# Autodesk Inventor assembly: Swerve-Drivetrain-2
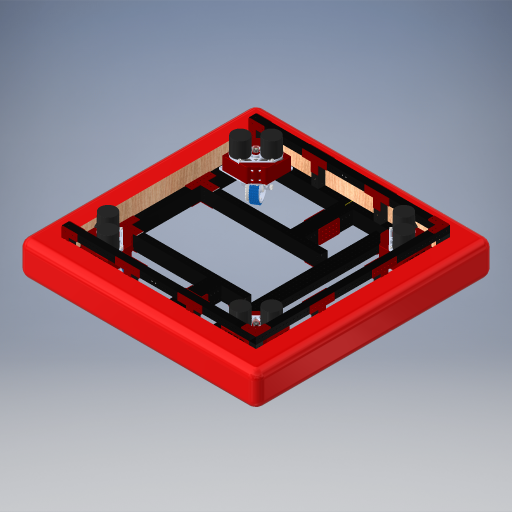
[picture p0: Inventor's stored thumbnail of the model, 512x512]
Saved by Autodesk Inventor 2024.2 (Build 282272000, 272)
## iProperties
Created: 2024-01-06
Part Number: Swerve-Drivetrain-2
Document SubType Name: Assembly
Designer: rohan
Author: rohan
## Documents named in this file (15)
- C:\Users\rohan\OneDrive - Hillsborough County Public Schools\Robotics\FIRST-Robotics-Competition\Crescendo\Minotaur-Crescendo-Robot\Swerve-Drivetrain.iam
- C:\Users\rohan\OneDrive - Hillsborough County Public Schools\Robotics\FIRST-Robotics-Competition\Crescendo\Minotaur-Crescendo-Robot\Motion\Swerve-Modules\MK3-Swerve-Module-Neos.iam
- C:\Users\rohan\OneDrive - Hillsborough County Public Schools\Robotics\FIRST-Robotics-Competition\Crescendo\Minotaur-Crescendo-Robot\Structure\Aluminum-Extrusions\2024-100-002-Front-Back-Extrusions.ipt
- C:\Users\rohan\OneDrive - Hillsborough County Public Schools\Robotics\FIRST-Robotics-Competition\Crescendo\Minotaur-Crescendo-Robot\Structure\Aluminum-Extrusions\2024-100-001-Left-Right-Extrusions.ipt
- C:\Users\rohan\OneDrive - Hillsborough County Public Schools\Robotics\FIRST-Robotics-Competition\Crescendo\Minotaur-Crescendo-Robot\Structure\Aluminum-Extrusions\2024-100-003-Middle-Extrusions.ipt
- C:\Users\rohan\OneDrive - Hillsborough County Public Schools\Robotics\FIRST-Robotics-Competition\Crescendo\Minotaur-Crescendo-Robot\Structure\Gussets\THRIFYBOT-L-Gusset.ipt
- C:\Users\rohan\OneDrive - Hillsborough County Public Schools\Robotics\FIRST-Robotics-Competition\Crescendo\Minotaur-Crescendo-Robot\Structure\Bumpers.ipt
- C:\Users\rohan\OneDrive - Hillsborough County Public Schools\Robotics\FIRST-Robotics-Competition\Crescendo\Minotaur-Crescendo-Robot\Structure\Aluminum-Extrusions\2024-100-007-Front-B-Tubing-Mount.ipt
- C:\Users\rohan\OneDrive - Hillsborough County Public Schools\Robotics\FIRST-Robotics-Competition\Crescendo\Minotaur-Crescendo-Robot\Structure\Gussets\THRIFYBOT-T-Gusset.ipt
- C:\Users\rohan\OneDrive - Hillsborough County Public Schools\Robotics\FIRST-Robotics-Competition\Crescendo\Minotaur-Crescendo-Robot\Structure\Gussets\Custom-Underside-T-Gusset.ipt
- C:\Users\rohan\OneDrive - Hillsborough County Public Schools\Robotics\FIRST-Robotics-Competition\Crescendo\Minotaur-Crescendo-Robot\Structure\Gussets\Custom-Underside-L-Gusset.ipt
- C:\Users\rohan\OneDrive - Hillsborough County Public Schools\Robotics\FIRST-Robotics-Competition\Crescendo\Minotaur-Crescendo-Robot\Structure\Aluminum-Extrusions\Superstructure-Mount.iam
- C:\Users\rohan\OneDrive - Hillsborough County Public Schools\Robotics\FIRST-Robotics-Competition\Crescendo\Minotaur-Crescendo-Robot\Structure\Gussets\3x5-Grid-Gusset.ipt
- C:\Users\rohan\OneDrive - Hillsborough County Public Schools\Robotics\FIRST-Robotics-Competition\Crescendo\Minotaur-Crescendo-Robot\Structure\Aluminum-Extrusions\2024-100-005-Climber-Mount.ipt
- C:\Users\rohan\OneDrive - Hillsborough County Public Schools\Robotics\FIRST-Robotics-Competition\Crescendo\Minotaur-Crescendo-Robot\Structure\Aluminum-Extrusions\2024-100-010-Climber-Support.ipt
## Components (33 placed, 14 different names)
1. MK3-Swerve-Module-Neos:1 [sub-assembly] — Mate:75, Mate:80, Mate:81
2. MK3-Swerve-Module-Neos:2 [sub-assembly] — Mate:74, Mate:82, Mate:83
3. MK3-Swerve-Module-Neos:3 [sub-assembly] — Mate:73, Mate:76, Mate:77
4. MK3-Swerve-Module-Neos:4 [sub-assembly] — Mate:72, Mate:78, Mate:79
5. 2024-100-001-Left-Right-Extrusions:1 — Mate:69, Flush:1, Flush:2, Mate:70, Flush:3, Flush:4, Mate:73, Mate:76, Mate:82, Flush:12, Flush:14, Flush:45, Mate:111, Flush:53, Flush:54, Mate:122, Flush:71
6. 2024-100-001-Left-Right-Extrusions:2 — Mate:71, Flush:5, Flush:6, Mate:79, Mate:81, Flush:10, Flush:16, Mate:99, Mate:106, Flush:51
7. 2024-100-002-Front-Back-Extrusions:1 — Mate:70, Flush:3, Flush:4, Mate:72, Mate:77, Mate:78, Mate:88, Mate:89, Flush:13, Flush:15, Flush:33, Mate:112
8. 2024-100-002-Front-Back-Extrusions:2 — Mate:69, Flush:1, Flush:2, Mate:71, Flush:5, Flush:6, Mate:74, Mate:75, Mate:80, Mate:83, Mate:86, Mate:87, Flush:9, Flush:11, Mate:98, Mate:101, Flush:38, Flush:40, Insert:1, Flush:43, Mate:105, Insert:2, Flush:55, Mate:123, Mate:124
9. THRIFYBOT-L-Gusset:1 — Mate:89, Flush:13, Flush:14
10. THRIFYBOT-L-Gusset:2 — Mate:88, Flush:15, Flush:16
11. THRIFYBOT-L-Gusset:3 — Mate:87, Flush:11, Flush:12
12. THRIFYBOT-L-Gusset:4 — Mate:86, Flush:9, Flush:10
13. Bumpers:1 — Mate:98, Mate:99, Flush:33
14. 2024-100-007-Front-B-Tubing-Mount:1 — Mate:100, Flush:34, Mate:101, Flush:35, Flush:39, Mate:103, Flush:40, Mate:107, Flush:48, Insert:3, Mate:121, Flush:70
15. 2024-100-007-Front-B-Tubing-Mount:2 — Mate:100, Flush:34, Flush:35, Flush:44, Flush:47, Insert:4
16. THRIFYBOT-T-Gusset:1 — Flush:36, Mate:102, Flush:37, Mate:103
17. THRIFYBOT-T-Gusset:2 — Flush:36, Mate:102, Flush:37, Flush:38, Flush:39, Insert:1
18. THRIFYBOT-T-Gusset:3 — Mate:105
19. THRIFYBOT-T-Gusset:4 — Flush:43, Flush:44, Insert:2
20. 2024-100-003-Middle-Extrusions:1 — Flush:45, Mate:106, Mate:107, Mate:108, Mate:109, Flush:46, Flush:49, Mate:110, Flush:50, Flush:52
21. Custom-Underside-T-Gusset:1 — Mate:108, Flush:48, Flush:49, Insert:3
22. Custom-Underside-T-Gusset:2 — Mate:109, Flush:46, Flush:47, Insert:4
23. Custom-Underside-L-Gusset:4 — Mate:111, Flush:52, Flush:53
24. Custom-Underside-L-Gusset:5 — Mate:110, Flush:50, Flush:51
25. Superstructure-Mount:1 [sub-assembly] — Mate:112, Flush:54, Flush:55
26. 3x5-Grid-Gusset:1 — Flush:56, Flush:57, Mate:113, Mate:117
27. 3x5-Grid-Gusset:2 — Flush:56, Flush:57, Mate:113, Flush:64, Insert:5
28. 2024-100-005-Climber-Mount:1 — Flush:60, Flush:61, Mate:115, Flush:64, Mate:117, Insert:5, Mate:122, Flush:71, Mate:124
29. 2024-100-010-Climber-Support:1 — Flush:60, Flush:61, Mate:115
30. 3x5-Grid-Gusset:3
31. 3x5-Grid-Gusset:4
32. 2024-100-005-Climber-Mount:2 — Flush:70, Mate:123
33. 2024-100-010-Climber-Support:2 — Mate:121
## Relationships (99: Flush 49, Mate 44, Insert 6)
- Mate:69: 2024-100-001-Left-Right-Extrusions:1 ↔ 2024-100-002-Front-Back-Extrusions:2
- Flush:1: 2024-100-001-Left-Right-Extrusions:1 ↔ 2024-100-002-Front-Back-Extrusions:2
- Flush:2: 2024-100-001-Left-Right-Extrusions:1 ↔ 2024-100-002-Front-Back-Extrusions:2
- Mate:70: 2024-100-001-Left-Right-Extrusions:1 ↔ 2024-100-002-Front-Back-Extrusions:1
- Flush:3: 2024-100-001-Left-Right-Extrusions:1 ↔ 2024-100-002-Front-Back-Extrusions:1
- Flush:4: 2024-100-001-Left-Right-Extrusions:1 ↔ 2024-100-002-Front-Back-Extrusions:1
- Mate:71: 2024-100-001-Left-Right-Extrusions:2 ↔ 2024-100-002-Front-Back-Extrusions:2
- Flush:5: 2024-100-001-Left-Right-Extrusions:2 ↔ 2024-100-002-Front-Back-Extrusions:2
- Flush:6: 2024-100-001-Left-Right-Extrusions:2 ↔ 2024-100-002-Front-Back-Extrusions:2
- Mate:72: MK3-Swerve-Module-Neos:4 ↔ 2024-100-002-Front-Back-Extrusions:1
- Mate:73: MK3-Swerve-Module-Neos:3 ↔ 2024-100-001-Left-Right-Extrusions:1
- Mate:74: MK3-Swerve-Module-Neos:2 ↔ 2024-100-002-Front-Back-Extrusions:2
- Mate:75: MK3-Swerve-Module-Neos:1 ↔ 2024-100-002-Front-Back-Extrusions:2
- Mate:76: MK3-Swerve-Module-Neos:3 ↔ 2024-100-001-Left-Right-Extrusions:1
- Mate:77: MK3-Swerve-Module-Neos:3 ↔ 2024-100-002-Front-Back-Extrusions:1
- Mate:78: MK3-Swerve-Module-Neos:4 ↔ 2024-100-002-Front-Back-Extrusions:1
- Mate:79: MK3-Swerve-Module-Neos:4 ↔ 2024-100-001-Left-Right-Extrusions:2
- Mate:80: MK3-Swerve-Module-Neos:1 ↔ 2024-100-002-Front-Back-Extrusions:2
- Mate:81: MK3-Swerve-Module-Neos:1 ↔ 2024-100-001-Left-Right-Extrusions:2
- Mate:82: MK3-Swerve-Module-Neos:2 ↔ 2024-100-001-Left-Right-Extrusions:1
- Mate:83: MK3-Swerve-Module-Neos:2 ↔ 2024-100-002-Front-Back-Extrusions:2
- Mate:86: 2024-100-002-Front-Back-Extrusions:2 ↔ THRIFYBOT-L-Gusset:4
- Mate:87: 2024-100-002-Front-Back-Extrusions:2 ↔ THRIFYBOT-L-Gusset:3
- Mate:88: 2024-100-002-Front-Back-Extrusions:1 ↔ THRIFYBOT-L-Gusset:2
- Mate:89: 2024-100-002-Front-Back-Extrusions:1 ↔ THRIFYBOT-L-Gusset:1
- Flush:9: 2024-100-002-Front-Back-Extrusions:2 ↔ THRIFYBOT-L-Gusset:4
- Flush:10: 2024-100-001-Left-Right-Extrusions:2 ↔ THRIFYBOT-L-Gusset:4
- Flush:11: 2024-100-002-Front-Back-Extrusions:2 ↔ THRIFYBOT-L-Gusset:3
- Flush:12: 2024-100-001-Left-Right-Extrusions:1 ↔ THRIFYBOT-L-Gusset:3
- Flush:13: 2024-100-002-Front-Back-Extrusions:1 ↔ THRIFYBOT-L-Gusset:1
- Flush:14: 2024-100-001-Left-Right-Extrusions:1 ↔ THRIFYBOT-L-Gusset:1
- Flush:15: 2024-100-002-Front-Back-Extrusions:1 ↔ THRIFYBOT-L-Gusset:2
- Flush:16: 2024-100-001-Left-Right-Extrusions:2 ↔ THRIFYBOT-L-Gusset:2
- Mate:98: 2024-100-002-Front-Back-Extrusions:2 ↔ Bumpers:1
- Mate:99: 2024-100-001-Left-Right-Extrusions:2 ↔ Bumpers:1
- Flush:33 (63.5 mm): 2024-100-002-Front-Back-Extrusions:1 ↔ Bumpers:1
- Mate:100 (254 mm): 2024-100-007-Front-B-Tubing-Mount:1 ↔ 2024-100-007-Front-B-Tubing-Mount:2
- Flush:34: 2024-100-007-Front-B-Tubing-Mount:1 ↔ 2024-100-007-Front-B-Tubing-Mount:2
- Mate:101: 2024-100-002-Front-Back-Extrusions:2 ↔ 2024-100-007-Front-B-Tubing-Mount:1
- Flush:35: 2024-100-007-Front-B-Tubing-Mount:1 ↔ 2024-100-007-Front-B-Tubing-Mount:2
- Flush:36: THRIFYBOT-T-Gusset:1 ↔ THRIFYBOT-T-Gusset:2
- Mate:102 (50.8 mm): THRIFYBOT-T-Gusset:1 ↔ THRIFYBOT-T-Gusset:2
- Flush:37: THRIFYBOT-T-Gusset:1 ↔ THRIFYBOT-T-Gusset:2
- Flush:38: 2024-100-002-Front-Back-Extrusions:2 ↔ THRIFYBOT-T-Gusset:2
- Flush:39: 2024-100-007-Front-B-Tubing-Mount:1 ↔ THRIFYBOT-T-Gusset:2
- Mate:103: 2024-100-007-Front-B-Tubing-Mount:1 ↔ THRIFYBOT-T-Gusset:1
- Flush:40: 2024-100-002-Front-Back-Extrusions:2 ↔ 2024-100-007-Front-B-Tubing-Mount:1
- Insert:1: 2024-100-002-Front-Back-Extrusions:2 ↔ THRIFYBOT-T-Gusset:2
- [Flush]: THRIFYBOT-T-Gusset:3 ↔ THRIFYBOT-T-Gusset:4
- [Mate] (50.8 mm): THRIFYBOT-T-Gusset:3 ↔ THRIFYBOT-T-Gusset:4
- [Flush]: THRIFYBOT-T-Gusset:3 ↔ THRIFYBOT-T-Gusset:4
- Flush:43: 2024-100-002-Front-Back-Extrusions:2 ↔ THRIFYBOT-T-Gusset:4
- Flush:44: 2024-100-007-Front-B-Tubing-Mount:2 ↔ THRIFYBOT-T-Gusset:4
- Mate:105: 2024-100-002-Front-Back-Extrusions:2 ↔ THRIFYBOT-T-Gusset:3
- Insert:2: 2024-100-002-Front-Back-Extrusions:2 ↔ THRIFYBOT-T-Gusset:4
- Flush:45: 2024-100-001-Left-Right-Extrusions:1 ↔ 2024-100-003-Middle-Extrusions:1
- Mate:106: 2024-100-001-Left-Right-Extrusions:2 ↔ 2024-100-003-Middle-Extrusions:1
- Mate:107: 2024-100-007-Front-B-Tubing-Mount:1 ↔ 2024-100-003-Middle-Extrusions:1
- Mate:108: 2024-100-003-Middle-Extrusions:1 ↔ Custom-Underside-T-Gusset:1
- Mate:109: 2024-100-003-Middle-Extrusions:1 ↔ Custom-Underside-T-Gusset:2
- Flush:46: 2024-100-003-Middle-Extrusions:1 ↔ Custom-Underside-T-Gusset:2
- Flush:47: 2024-100-007-Front-B-Tubing-Mount:2 ↔ Custom-Underside-T-Gusset:2
- Flush:48: 2024-100-007-Front-B-Tubing-Mount:1 ↔ Custom-Underside-T-Gusset:1
- Flush:49: 2024-100-003-Middle-Extrusions:1 ↔ Custom-Underside-T-Gusset:1
- Insert:3: 2024-100-007-Front-B-Tubing-Mount:1 ↔ Custom-Underside-T-Gusset:1
- Insert:4: 2024-100-007-Front-B-Tubing-Mount:2 ↔ Custom-Underside-T-Gusset:2
- Mate:110: 2024-100-003-Middle-Extrusions:1 ↔ Custom-Underside-L-Gusset:5
- Flush:50: 2024-100-003-Middle-Extrusions:1 ↔ Custom-Underside-L-Gusset:5
- Flush:51: 2024-100-001-Left-Right-Extrusions:2 ↔ Custom-Underside-L-Gusset:5
- Mate:111: 2024-100-001-Left-Right-Extrusions:1 ↔ Custom-Underside-L-Gusset:4
- Flush:52: 2024-100-003-Middle-Extrusions:1 ↔ Custom-Underside-L-Gusset:4
- Flush:53: 2024-100-001-Left-Right-Extrusions:1 ↔ Custom-Underside-L-Gusset:4
- Mate:112: 2024-100-002-Front-Back-Extrusions:1 ↔ Superstructure-Mount:1
- Flush:54: 2024-100-001-Left-Right-Extrusions:1 ↔ Superstructure-Mount:1
- Flush:55: 2024-100-002-Front-Back-Extrusions:2 ↔ Superstructure-Mount:1
- Flush:56: 3x5-Grid-Gusset:1 ↔ 3x5-Grid-Gusset:2
- Flush:57: 3x5-Grid-Gusset:1 ↔ 3x5-Grid-Gusset:2
- Mate:113 (50.8 mm): 3x5-Grid-Gusset:1 ↔ 3x5-Grid-Gusset:2
- Flush:60: 2024-100-005-Climber-Mount:1 ↔ 2024-100-010-Climber-Support:1
- Flush:61: 2024-100-005-Climber-Mount:1 ↔ 2024-100-010-Climber-Support:1
- Mate:115: 2024-100-005-Climber-Mount:1 ↔ 2024-100-010-Climber-Support:1
- Flush:64: 3x5-Grid-Gusset:2 ↔ 2024-100-005-Climber-Mount:1
- Mate:117: 3x5-Grid-Gusset:1 ↔ 2024-100-005-Climber-Mount:1
- Insert:5: 3x5-Grid-Gusset:2 ↔ 2024-100-005-Climber-Mount:1
- [Flush]: 3x5-Grid-Gusset:3 ↔ 3x5-Grid-Gusset:4
- [Flush]: 3x5-Grid-Gusset:3 ↔ 3x5-Grid-Gusset:4
- [Mate] (50.8 mm): 3x5-Grid-Gusset:3 ↔ 3x5-Grid-Gusset:4
- [Flush]: 2024-100-005-Climber-Mount:2 ↔ 2024-100-010-Climber-Support:2
- [Flush]: 2024-100-005-Climber-Mount:2 ↔ 2024-100-010-Climber-Support:2
- [Mate]: 2024-100-005-Climber-Mount:2 ↔ 2024-100-010-Climber-Support:2
- [Flush]: 3x5-Grid-Gusset:4 ↔ 2024-100-005-Climber-Mount:2
- [Mate]: 3x5-Grid-Gusset:3 ↔ 2024-100-005-Climber-Mount:2
- [Insert]: 3x5-Grid-Gusset:4 ↔ 2024-100-005-Climber-Mount:2
- Mate:121: 2024-100-007-Front-B-Tubing-Mount:1 ↔ 2024-100-010-Climber-Support:2
- Flush:70: 2024-100-007-Front-B-Tubing-Mount:1 ↔ 2024-100-005-Climber-Mount:2
- Mate:122: 2024-100-001-Left-Right-Extrusions:1 ↔ 2024-100-005-Climber-Mount:1
- Flush:71: 2024-100-001-Left-Right-Extrusions:1 ↔ 2024-100-005-Climber-Mount:1
- Mate:123 (304.8 mm): 2024-100-002-Front-Back-Extrusions:2 ↔ 2024-100-005-Climber-Mount:2
- Mate:124 (304.8 mm): 2024-100-002-Front-Back-Extrusions:2 ↔ 2024-100-005-Climber-Mount:1
## Named parameters: d320_d312 = 0 mm, d321_d313 = 50.8 mm, d322_d314 = 0 mm, d377_d362 = 0 mm, d378_d363 = 0 mm, d379_d364 = 50.8 mm, d380_d368 = 0 mm, d381_d369 = 0 mm, d382_d370 = 0 mm, d383_d374 = 0 mm, d384_d375 = 0 mm, d385_d376 = 0 mm
